# Autodesk Inventor assembly: bw_ass_1
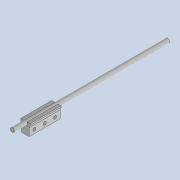
[picture p0: Inventor's stored thumbnail of the model, 180x180]
Saved by Autodesk Inventor 2020 (Build 240168000, 168)
## iProperties
Created: 2021-09-10
Part Number: bw_ass_1
Document SubType Name: Assembly
Designer: Shuang Peng
Author: Shuang Peng
## Documents named in this file (3)
- D:\projects-3\torque fb tip\hardware\tip_3\bw_ass_1.iam
- D:\projects-3\torque fb tip\hardware\tip_3\bw_tube_0.8_1.6.ipt
- D:\projects-3\torque fb tip\hardware\tip_3\bw_hl_1.ipt
## Components (2 placed, 2 different names)
1. bw_tube_0.8_1.6:1 — Insert:1
2. bw_hl_1:1 — Insert:1
## Relationships (1: Insert 1)
- Insert:1: bw_tube_0.8_1.6:1 ↔ bw_hl_1:1
